# Autodesk Inventor assembly: RC car
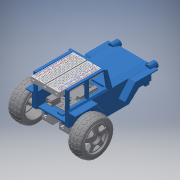
[picture p0: Inventor's stored thumbnail of the model, 180x180]
Saved by Autodesk Inventor 2019 (Build 230136000, 136)
## iProperties
Created: 2020-12-08
Part Number: RC car
Document SubType Name: Assembly
Designer: saeva
Author: saeva
## Documents named in this file (7)
- C:\Users\saeva\OneDrive\Desktop\RC car.iam
- C:\Users\saeva\Downloads\arduino uno.iam
- C:\Users\saeva\OneDrive\Desktop\HalfBreadboard.ipt
- C:\Users\saeva\OneDrive\Desktop\Wheel D65x25.ipt
- C:\Users\saeva\OneDrive\Desktop\motor\3-6V DC Gearbox Electromotor.iam
- C:\Users\saeva\OneDrive\Desktop\chasis.ipt
- C:\Users\saeva\OneDrive\Desktop\ballbearing.ipt
## Components (8 placed, 6 different names)
1. arduino uno:1 [sub-assembly] — Flush:1
2. HalfBreadboard:1 — Flush:2, Mate:15, Mate:16
3. Wheel D65x25:3
4. 3-6V DC Gearbox Electromotor:2 [sub-assembly] — Mate:17, Mate:22, Flush:3
5. chasis:1 — Flush:1, Flush:2, Mate:15, Mate:16, Mate:17, Mate:21, Mate:22, Mate:23, Flush:3, Flush:4, Mate:24
6. Wheel D65x25:4
7. 3-6V DC Gearbox Electromotor:3 [sub-assembly] — Mate:21, Mate:23, Flush:4
8. ballbearing:1 — Mate:24
## Relationships (15: Mate 11, Flush 4)
- [Mate]: Wheel D65x25:3 ↔ 3-6V DC Gearbox Electromotor:2
- [Mate]: Wheel D65x25:3 ↔ 3-6V DC Gearbox Electromotor:2
- Flush:1: arduino uno:1 ↔ chasis:1
- Flush:2: HalfBreadboard:1 ↔ chasis:1
- Mate:15: HalfBreadboard:1 ↔ chasis:1
- Mate:16: HalfBreadboard:1 ↔ chasis:1
- Mate:17: 3-6V DC Gearbox Electromotor:2 ↔ chasis:1
- [Mate]: Wheel D65x25:4 ↔ 3-6V DC Gearbox Electromotor:3
- [Mate]: Wheel D65x25:4 ↔ 3-6V DC Gearbox Electromotor:3
- Mate:21: chasis:1 ↔ 3-6V DC Gearbox Electromotor:3
- Mate:22: 3-6V DC Gearbox Electromotor:2 ↔ chasis:1
- Mate:23: chasis:1 ↔ 3-6V DC Gearbox Electromotor:3
- Flush:3: 3-6V DC Gearbox Electromotor:2 ↔ chasis:1
- Flush:4: chasis:1 ↔ 3-6V DC Gearbox Electromotor:3
- Mate:24: chasis:1 ↔ ballbearing:1
## Named parameters: d7_d3 = 0 mm, d8_d4 = 0 mm, d28_d7_d3 = 0 mm, d29_d8_d4 = 0 mm
